# Autodesk Inventor assembly: 276-1489
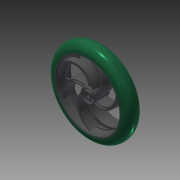
[picture p0: Inventor's stored thumbnail of the model, 180x180]
Saved by Autodesk Inventor 2016 SP2 (Build 200236200, 236)
## iProperties
Company: Innovation First, Inc.
Created: 2007-08-25
Part Number: 276-1489
Description: STEP AP203
Document SubType Name: Assembly
Designer: Jacob
Sending System: SolidWorks 2006052
Preprocessor: SwSTEP 2.0
Title: VEX-MEDIUM-WHEEL.STEP
Author: Jacob (7842)
Revision Number: ANY
## Documents named in this file (3)
- D:\Users\Owner\Desktop\Inventor Files\VEX Parts\Imperial\Motion\4 inch High Traction Wheel.iam
- D:\Users\Owner\Desktop\Inventor Files\VEX Parts\Imperial\Motion\Components\MEDIUM-WHEEL-HUB.ipt
- D:\Users\Owner\Desktop\Inventor Files\VEX Parts\Imperial\Motion\Components\VEX-4INCH-HIGHTRACTION-TIRE.iam
## Components (2 placed, 2 different names)
1. MEDIUM-WHEEL-HUB_1 — Mate:1, Angle:1, Insert:1
2. VEX-4INCH-HIGHTRACTION-TIRE:1 [sub-assembly] — Mate:1, Angle:1, Insert:1
## Relationships (3: Mate 1, Angle 1, Insert 1)
- Mate:1: MEDIUM-WHEEL-HUB_1 ↔ VEX-4INCH-HIGHTRACTION-TIRE:1
- Angle:1 (0 deg): MEDIUM-WHEEL-HUB_1 ↔ VEX-4INCH-HIGHTRACTION-TIRE:1
- Insert:1 (-0.381 mm): MEDIUM-WHEEL-HUB_1 ↔ VEX-4INCH-HIGHTRACTION-TIRE:1
